# Autodesk Inventor assembly: NEW_COVER_220DET_COMPLETE
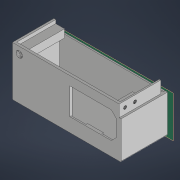
[picture p0: Inventor's stored thumbnail of the model, 180x180]
Saved by Autodesk Inventor 2021 (Build 250183000, 183)
## iProperties
Created: 2020-07-15
Part Number: NEW_COVER_220DET_COMPLETE
Document SubType Name: Assembly
Designer: erwin
Author: erwin
## Documents named in this file (3)
- D:\OneDrive\Projects\RepRap\_Parts\New\PSU cover\NEW_COVER_220DET_COMPLETE.iam
- D:\OneDrive\Projects\RepRap\_Parts\New\PSU cover\NEW_COVER_220DET.ipt
- D:\OneDrive\Projects\RepRap\_Parts\New\PSU cover\NEW_COVER_220DET_SMALL_COVER.ipt
## Components (2 placed, 2 different names)
1. NEW_COVER_220DET:1 — Flush:1, Flush:2
2. NEW_COVER_220DET_SMALL_COVER:1 — Flush:1, Flush:2
## Relationships (2: Flush 2)
- Flush:1: NEW_COVER_220DET:1 ↔ NEW_COVER_220DET_SMALL_COVER:1
- Flush:2: NEW_COVER_220DET:1 ↔ NEW_COVER_220DET_SMALL_COVER:1
